# Autodesk Inventor assembly: assembly_robot_arm
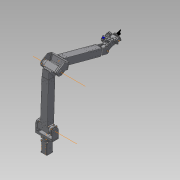
[picture p0: Inventor's stored thumbnail of the model, 180x180]
Saved by Autodesk Inventor 2017 (Build 210142000, 142)
## iProperties
Part Number: assembly_robot_arm
Material: Generisch
Document SubType Name: Assembly
Designer: Max
Author: Max
## Documents named in this file (8)
- C:\Users\Max\Desktop\SENAI\robot_arm_new\assembly_robot_arm.iam
- C:\Users\Max\Desktop\SENAI\robot_arm_new\h54-200-s500-r.ipt
- C:\Users\Max\Desktop\SENAI\robot_arm_new\dynamixel_pro_frame.iam
- C:\Users\Max\Desktop\SENAI\robot_arm_new\assembly_arm_1.iam
- C:\Users\Max\Desktop\SENAI\robot_arm_new\assembly_arm_2.iam
- C:\Users\Max\Desktop\SENAI\robot_arm_new\frame_mx108.ipt
- C:\Users\Max\Desktop\SENAI\robot_arm_new\assembly_hand.iam
- C:\Users\Max\Desktop\SENAI\robot_arm_new\Pointing_Finger.ipt
## Components (7 placed, 7 different names)
1. h54-200-s500-r:3 — Passend:6, Passend:7, Passend:8, Passend:9, Passend:10, Winkel:3
2. dynamixel_pro_frame:1 [sub-assembly] — Passend:9, Passend:10, Passend:11, Winkel:3, Passend:24
3. assembly_arm_1:1 [sub-assembly] — Passend:11, Passend:14, Passend:21, Passend:23, Passend:24, Passend:25, Passend:28
4. assembly_arm_2:1 [sub-assembly] — Passend:14, Passend:16, Passend:17, Passend:25, Passend:28
5. frame_mx108:1 — Passend:16, Passend:17, Passend:18, Passend:19
6. assembly_hand:1 [sub-assembly] — Passend:18, Passend:19, Passend:26, Passend:27
7. Pointing_Finger:1 — Passend:26, Passend:27
## Relationships (19: Mate 18, Angle 1)
- Passend:6 [Mate]: h54-200-s500-r:3
- Passend:7 [Mate]: h54-200-s500-r:3
- Passend:8 [Mate]: h54-200-s500-r:3
- Passend:9 [Mate]: h54-200-s500-r:3 ↔ dynamixel_pro_frame:1
- Passend:10 [Mate]: h54-200-s500-r:3 ↔ dynamixel_pro_frame:1
- Passend:11 [Mate]: dynamixel_pro_frame:1 ↔ assembly_arm_1:1
- Passend:14 [Mate]: assembly_arm_1:1 ↔ assembly_arm_2:1
- Passend:16 [Mate]: assembly_arm_2:1 ↔ frame_mx108:1
- Passend:17 [Mate]: assembly_arm_2:1 ↔ frame_mx108:1
- Passend:18 [Mate]: frame_mx108:1 ↔ assembly_hand:1
- Passend:19 [Mate]: frame_mx108:1 ↔ assembly_hand:1
- Passend:21 [Mate]: assembly_arm_1:1
- Passend:23 [Mate]: assembly_arm_1:1
- Winkel:3 [Angle] (0 deg): h54-200-s500-r:3 ↔ dynamixel_pro_frame:1
- Passend:24 [Mate]: dynamixel_pro_frame:1 ↔ assembly_arm_1:1
- Passend:25 [Mate]: assembly_arm_1:1 ↔ assembly_arm_2:1
- Passend:26 [Mate]: assembly_hand:1 ↔ Pointing_Finger:1
- Passend:27 [Mate]: assembly_hand:1 ↔ Pointing_Finger:1
- Passend:28 [Mate]: assembly_arm_1:1 ↔ assembly_arm_2:1
